# Autodesk Inventor assembly: ASY NDM 11.0 перегородка
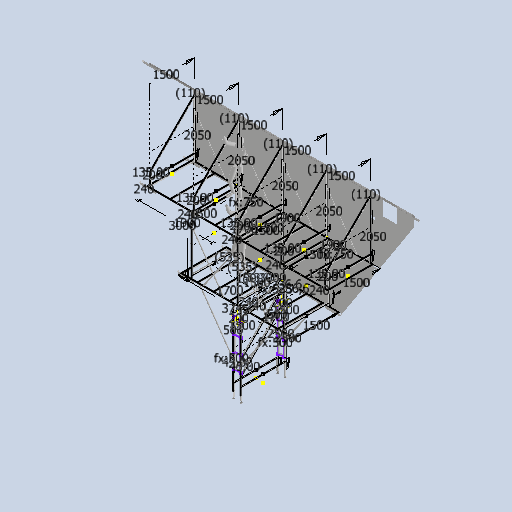
[picture p0: Inventor's stored thumbnail of the model, 512x512]
Saved by Autodesk Inventor 2025 (Build 290162010, 162A)
## iProperties
Created: 2024-05-21
Part Number: ASY NDM 11.0 перегородка
Document SubType Name: Assembly
Designer: admin
Author: admin
## Documents named in this file (18)
- C:\Users\user\YandexDisk\домашниий пк\Inventor\Nadyim\CAD\Перегородка\ASY NDM 11.0 перегородка.iam
- C:\Users\user\YandexDisk\домашниий пк\Inventor\Nadyim\CAD\dummi\human 01\ч ASY human dummy 01.iam
- C:\Users\user\YandexDisk\домашниий пк\Inventor\Nadyim\CAD\Перегородка\NDM 11.012 лист 12.ipt
- C:\Users\user\YandexDisk\домашниий пк\Inventor\Nadyim\CAD\Перегородка\ASY NDM 11.020 перегородка рама 1 горизонт.iam
- C:\Users\user\YandexDisk\домашниий пк\Inventor\Nadyim\CAD\Перегородка\ASY NDM 11.030 перегородка рама 2 горизонт.iam
- C:\Users\user\YandexDisk\домашниий пк\Inventor\Nadyim\CAD\Перегородка\ASY NDM 11.023 перегородка рама 1 вертикал.iam
- C:\Users\user\YandexDisk\домашниий пк\Inventor\Nadyim\CAD\Screwjack pilar\ASY NDM 14.0 Screwjack pillar 1.iam
- C:\Users\user\YandexDisk\домашниий пк\Inventor\Nadyim\CAD\NDM 7.4 bracket bottom mother.ipt
- C:\Users\user\YandexDisk\домашниий пк\Inventor\Nadyim\CAD\Перегородка\ASY NDM 11.040 рама 3 вертикал угол.iam
- C:\Users\user\YandexDisk\домашниий пк\Inventor\Nadyim\CAD\Перегородка\ASY NDM 11.050 перегородка рама 2 вертикал.iam
- C:\Users\user\YandexDisk\домашниий пк\Inventor\Nadyim\CAD\Перегородка\ASY NDM 11.043 верхняя перемычка.ipt
- C:\Users\user\YandexDisk\домашниий пк\Inventor\Nadyim\CAD\Перегородка\ASY NDM 11.025 перегородка рама 1.1  вертикал.iam
- C:\Users\user\YandexDisk\домашниий пк\Inventor\Nadyim\CAD\Перегородка\ASY NDM 11.035 укосина.iam
- C:\Users\user\YandexDisk\домашниий пк\Inventor\Nadyim\CAD\Перегородка\ASY NDM 11.036 укосина.iam
- C:\Users\user\YandexDisk\домашниий пк\Inventor\Nadyim\CAD\Перегородка\ASY NDM 11.037 упор.iam
- C:\Users\user\YandexDisk\домашниий пк\Inventor\Nadyim\CAD\Перегородка\NDM 11.013 лист 131.ipt
- C:\Users\user\YandexDisk\домашниий пк\Inventor\Nadyim\CAD\Перегородка\NDM 11.014 лист 141.ipt
- C:\Users\user\YandexDisk\домашниий пк\Inventor\Nadyim\CAD\Перегородка\NDM 11.015 лист 15.ipt
## Components (62 placed, 17 different names)
1. ч ASY human dummy 01:1 [sub-assembly]
2. ч ASY human dummy 01:2 [sub-assembly]
3. ASY NDM 11.020 перегородка рама 1 горизонт:1 [sub-assembly] — Mate:3, Flush:4, Flush:6, Flush:8, Mate:8, Flush:10, Mate:25, Mate:31, Mate:34, Mate:35, Mate:36, Mate:68, Mate:72, Mate:77, Mate:80, Mate:82, Flush:14, Mate:84, Mate:85, Mate:88, Mate:89, Mate:96, Mate:97
4. ASY NDM 11.030 перегородка рама 2 горизонт:1 [sub-assembly] — Rigid:16, Mate:6, Flush:7, Flush:8, Mate:10, Mate:43, Mate:49, Mate:61, Mate:62, Mate:83, Flush:15, Mate:86, Mate:87, Mate:107, Mate:108
5. ASY NDM 11.030 перегородка рама 2 горизонт:2 [sub-assembly] — Rigid:16, Mate:7, Mate:40, Mate:50, Mate:51, Mate:56, Mate:92, Mate:93, Mate:94, Mate:95, Mate:104, Mate:105, Mate:112, Mate:113
6. ASY NDM 11.023 перегородка рама 1 вертикал:1 [sub-assembly] — Mate:3, Flush:4, Rigid:19, Rigid:20, Mate:5, Flush:5, Rigid:21, Flush:12, Mate:15, Mate:16, Mate:18, Mate:19, Mate:66, Mate:67, Mate:73, Mate:74
7. ASY NDM 14.0 Screwjack pillar 1:1 [sub-assembly] — Rigid:17, Rigid:20, Mate:4
8. NDM 7.4 bracket bottom mother:1 — Rigid:17
9. ASY NDM 14.0 Screwjack pillar 1:2 [sub-assembly] — Rigid:19
10. NDM 7.4 bracket bottom mother:2
11. ASY NDM 11.023 перегородка рама 1 вертикал:2 [sub-assembly] — Rigid:21, Rigid:28, Rigid:29, Mate:17, Mate:75, Mate:76, Mate:78, Mate:79
12. ASY NDM 11.050 перегородка рама 2 вертикал:1 [sub-assembly] — Mate:8, Flush:10, Mate:9, Mate:10, Rigid:22, Rigid:23, Mate:29, Mate:30, Mate:32, Mate:33, Mate:106, Mate:109
13. ASY NDM 11.050 перегородка рама 2 вертикал:2 [sub-assembly] — Rigid:22, Mate:37
14. ASY NDM 11.050 перегородка рама 2 вертикал:3 [sub-assembly] — Rigid:23, Mate:110, Mate:111, Mate:114
15. ASY NDM 11.043 верхняя перемычка:1 — Rigid:31, Mate:90, Mate:91, Mate:101, Mate:102
16. ASY NDM 11.043 верхняя перемычка:2 — Rigid:30, Rigid:31, Rigid:32, Mate:98, Mate:99
17. ASY NDM 14.0 Screwjack pillar 1:3 [sub-assembly] — Rigid:28
18. NDM 7.4 bracket bottom mother:3
19. ASY NDM 14.0 Screwjack pillar 1:4 [sub-assembly] — Rigid:29
20. NDM 7.4 bracket bottom mother:4
21. ASY NDM 11.025 перегородка рама 1.1  вертикал:1 [sub-assembly] — Flush:12, Mate:15, Mate:16
22. ASY NDM 11.025 перегородка рама 1.1  вертикал:2 [sub-assembly] — Mate:17, Mate:18, Mate:19
23. ASY NDM 11.035 укосина:2 [sub-assembly] — Mate:25, Mate:110, Mate:111
24. ASY NDM 11.035 укосина:3 [sub-assembly] — Mate:44, Mate:45, Mate:50
25. ASY NDM 11.035 укосина:4 [sub-assembly] — Mate:41, Mate:42, Mate:43
26. ASY NDM 11.035 укосина:5 [sub-assembly] — Mate:29, Mate:30, Mate:31
27. ASY NDM 11.036 укосина:1 [sub-assembly] — Mate:32, Mate:33, Mate:34
28. ASY NDM 11.036 укосина:2 [sub-assembly] — Mate:35, Mate:36, Mate:37
29. ASY NDM 11.036 укосина:3 [sub-assembly] — Mate:38, Mate:39, Mate:40
30. ASY NDM 11.035 укосина:6 [sub-assembly] — Mate:51, Mate:52, Mate:53
31. ASY NDM 11.035 укосина:7 [sub-assembly] — Mate:46, Mate:47, Mate:48, Mate:49
32. ASY NDM 11.036 укосина:4 [sub-assembly] — Mate:54, Mate:55, Mate:56
33. ASY NDM 11.036 укосина:5 [sub-assembly] — Mate:57, Mate:58, Mate:62
34. ASY NDM 11.036 укосина:6 [sub-assembly] — Mate:59, Mate:60, Mate:61
35. ASY NDM 11.043 верхняя перемычка:3 — Rigid:32
36. ASY NDM 11.035 укосина:8 [sub-assembly] — Mate:66, Mate:67, Mate:68
37. ASY NDM 11.035 укосина:9 [sub-assembly] — Mate:72, Mate:73, Mate:74
38. ASY NDM 11.035 укосина:10 [sub-assembly] — Mate:75, Mate:76, Mate:77
39. ASY NDM 11.035 укосина:11 [sub-assembly] — Mate:78, Mate:79, Mate:80
40. ASY NDM 11.037 упор:1 [sub-assembly]
41. ASY NDM 11.037 упор:2 [sub-assembly] — Mate:83, Flush:15, Flush:16
42. ASY NDM 11.037 упор:3 [sub-assembly] — Mate:82, Flush:14, Flush:17
43. ASY NDM 11.037 упор:4 [sub-assembly] — Mate:84, Mate:85, Flush:17
44. ASY NDM 11.037 упор:5 [sub-assembly] — Mate:86, Mate:87, Flush:16
45. ASY NDM 11.037 упор:6 [sub-assembly] — Mate:92, Mate:94, Flush:19, Flush:21
46. ASY NDM 11.037 упор:7 [sub-assembly] — Mate:93, Mate:95, Flush:19
47. ASY NDM 11.037 упор:8 [sub-assembly] — Mate:89, Mate:96, Flush:18, Flush:20, Flush:21
48. ASY NDM 11.037 упор:9 [sub-assembly] — Mate:88, Mate:97, Flush:18
49. ASY NDM 11.037 упор:10 [sub-assembly] — Mate:90, Mate:91, Flush:20
50. NDM 11.013 лист 131:1 — Mate:101, Mate:102, Mate:103
51. NDM 11.014 лист 141:1 — Mate:104, Mate:105, Mate:106
52. NDM 11.014 лист 141:2 — Mate:107, Mate:108, Mate:109
53. NDM 11.015 лист 15:1 — Mate:112, Mate:113, Mate:114
54. ASY NDM 11.040 рама 3 вертикал угол:1 [sub-assembly] — Mate:6, Flush:7, Flush:9, Mate:38, Mate:39, Mate:41, Mate:42, Rigid:30
55. ASY NDM 11.040 рама 3 вертикал угол:2 [sub-assembly] — Mate:46, Mate:47, Mate:48, Mate:57, Mate:58
56. ASY NDM 11.040 рама 3 вертикал угол:3 [sub-assembly] — Mate:44, Mate:45, Mate:54, Mate:55
57. ASY NDM 11.040 рама 3 вертикал угол:4 [sub-assembly] — Mate:59, Mate:60
58. ASY NDM 11.040 рама 3 вертикал угол:5 [sub-assembly] — Mate:52, Mate:53, Mate:100, Mate:103
59. NDM 11.012 лист 12:5 — Mate:98, Mate:99, Mate:100
60. NDM 11.012 лист 12:6
61. NDM 11.012 лист 12:7
62. NDM 11.012 лист 12:8
## Component patterns: (5 elements, first: ASY NDM 11.040 рама 3 вертикал угол:1), (4 elements, first: NDM 11.012 лист 12:5)
## Relationships (126: Mate 94, Flush 17, WeldJoint 15)
- Rigid:16 [WeldJoint]: ASY NDM 11.030 перегородка рама 2 горизонт:1 ↔ ASY NDM 11.030 перегородка рама 2 горизонт:2
- Mate:3: ASY NDM 11.020 перегородка рама 1 горизонт:1 ↔ ASY NDM 11.023 перегородка рама 1 вертикал:1
- Flush:4: ASY NDM 11.020 перегородка рама 1 горизонт:1 ↔ ASY NDM 11.023 перегородка рама 1 вертикал:1
- Rigid:17 [WeldJoint] (40 mm): ASY NDM 14.0 Screwjack pillar 1:1 ↔ NDM 7.4 bracket bottom mother:1
- [WeldJoint] (40 mm): ASY NDM 14.0 Screwjack pillar 1:2 ↔ NDM 7.4 bracket bottom mother:2
- Rigid:19 [WeldJoint]: ASY NDM 11.023 перегородка рама 1 вертикал:1 ↔ ASY NDM 14.0 Screwjack pillar 1:2
- Rigid:20 [WeldJoint]: ASY NDM 11.023 перегородка рама 1 вертикал:1 ↔ ASY NDM 14.0 Screwjack pillar 1:1
- Mate:4: ASY NDM 14.0 Screwjack pillar 1:1
- Mate:5 (100 mm): ASY NDM 11.023 перегородка рама 1 вертикал:1
- Flush:5: ASY NDM 11.023 перегородка рама 1 вертикал:1
- Flush:6: ASY NDM 11.020 перегородка рама 1 горизонт:1
- Mate:6: ASY NDM 11.030 перегородка рама 2 горизонт:1 ↔ ASY NDM 11.040 рама 3 вертикал угол:1
- Flush:7: ASY NDM 11.030 перегородка рама 2 горизонт:1 ↔ ASY NDM 11.040 рама 3 вертикал угол:1
- Rigid:21 [WeldJoint] (204 mm): ASY NDM 11.023 перегородка рама 1 вертикал:1 ↔ ASY NDM 11.023 перегородка рама 1 вертикал:2
- Flush:8: ASY NDM 11.020 перегородка рама 1 горизонт:1 ↔ ASY NDM 11.030 перегородка рама 2 горизонт:1
- Flush:9: ASY NDM 11.040 рама 3 вертикал угол:1
- Mate:7: ASY NDM 11.030 перегородка рама 2 горизонт:2
- Mate:8 (2 mm): ASY NDM 11.020 перегородка рама 1 горизонт:1 ↔ ASY NDM 11.050 перегородка рама 2 вертикал:1
- Flush:10: ASY NDM 11.020 перегородка рама 1 горизонт:1 ↔ ASY NDM 11.050 перегородка рама 2 вертикал:1
- Mate:9: ASY NDM 11.050 перегородка рама 2 вертикал:1
- Mate:10 (2 mm): ASY NDM 11.030 перегородка рама 2 горизонт:1 ↔ ASY NDM 11.050 перегородка рама 2 вертикал:1
- Rigid:22 [WeldJoint] (1490 mm): ASY NDM 11.050 перегородка рама 2 вертикал:1 ↔ ASY NDM 11.050 перегородка рама 2 вертикал:2
- Rigid:23 [WeldJoint] (1530 mm): ASY NDM 11.050 перегородка рама 2 вертикал:1 ↔ ASY NDM 11.050 перегородка рама 2 вертикал:3
- [WeldJoint] (40 mm): ASY NDM 14.0 Screwjack pillar 1:3 ↔ NDM 7.4 bracket bottom mother:3
- [WeldJoint] (40 mm): ASY NDM 14.0 Screwjack pillar 1:4 ↔ NDM 7.4 bracket bottom mother:4
- Rigid:28 [WeldJoint]: ASY NDM 11.023 перегородка рама 1 вертикал:2 ↔ ASY NDM 14.0 Screwjack pillar 1:3
- Rigid:29 [WeldJoint]: ASY NDM 11.023 перегородка рама 1 вертикал:2 ↔ ASY NDM 14.0 Screwjack pillar 1:4
- Flush:12: ASY NDM 11.023 перегородка рама 1 вертикал:1 ↔ ASY NDM 11.025 перегородка рама 1.1  вертикал:1
- Mate:15: ASY NDM 11.023 перегородка рама 1 вертикал:1 ↔ ASY NDM 11.025 перегородка рама 1.1  вертикал:1
- Mate:16 (100 mm): ASY NDM 11.023 перегородка рама 1 вертикал:1 ↔ ASY NDM 11.025 перегородка рама 1.1  вертикал:1
- Mate:17: ASY NDM 11.023 перегородка рама 1 вертикал:2 ↔ ASY NDM 11.025 перегородка рама 1.1  вертикал:2
- Mate:18 (100 mm): ASY NDM 11.023 перегородка рама 1 вертикал:1 ↔ ASY NDM 11.025 перегородка рама 1.1  вертикал:2
- Mate:19: ASY NDM 11.023 перегородка рама 1 вертикал:1 ↔ ASY NDM 11.025 перегородка рама 1.1  вертикал:2
- Mate:25: ASY NDM 11.020 перегородка рама 1 горизонт:1 ↔ ASY NDM 11.035 укосина:2
- Mate:29: ASY NDM 11.050 перегородка рама 2 вертикал:1 ↔ ASY NDM 11.035 укосина:5
- Mate:30: ASY NDM 11.050 перегородка рама 2 вертикал:1 ↔ ASY NDM 11.035 укосина:5
- Mate:31: ASY NDM 11.020 перегородка рама 1 горизонт:1 ↔ ASY NDM 11.035 укосина:5
- Mate:32: ASY NDM 11.050 перегородка рама 2 вертикал:1 ↔ ASY NDM 11.036 укосина:1
- Mate:33: ASY NDM 11.050 перегородка рама 2 вертикал:1 ↔ ASY NDM 11.036 укосина:1
- Mate:34: ASY NDM 11.020 перегородка рама 1 горизонт:1 ↔ ASY NDM 11.036 укосина:1
- Mate:35: ASY NDM 11.020 перегородка рама 1 горизонт:1 ↔ ASY NDM 11.036 укосина:2
- Mate:36: ASY NDM 11.020 перегородка рама 1 горизонт:1 ↔ ASY NDM 11.036 укосина:2
- Mate:37: ASY NDM 11.050 перегородка рама 2 вертикал:2 ↔ ASY NDM 11.036 укосина:2
- Mate:38: ASY NDM 11.036 укосина:3 ↔ ASY NDM 11.040 рама 3 вертикал угол:1
- Mate:39: ASY NDM 11.036 укосина:3 ↔ ASY NDM 11.040 рама 3 вертикал угол:1
- Mate:40: ASY NDM 11.030 перегородка рама 2 горизонт:2 ↔ ASY NDM 11.036 укосина:3
- Mate:41: ASY NDM 11.035 укосина:4 ↔ ASY NDM 11.040 рама 3 вертикал угол:1
- Mate:42: ASY NDM 11.035 укосина:4 ↔ ASY NDM 11.040 рама 3 вертикал угол:1
- Mate:43: ASY NDM 11.030 перегородка рама 2 горизонт:1 ↔ ASY NDM 11.035 укосина:4
- Mate:44: ASY NDM 11.035 укосина:3 ↔ ASY NDM 11.040 рама 3 вертикал угол:3
- Mate:45: ASY NDM 11.035 укосина:3 ↔ ASY NDM 11.040 рама 3 вертикал угол:3
- Mate:46: ASY NDM 11.035 укосина:7 ↔ ASY NDM 11.040 рама 3 вертикал угол:2
- Mate:47: ASY NDM 11.035 укосина:7 ↔ ASY NDM 11.040 рама 3 вертикал угол:2
- Mate:48: ASY NDM 11.035 укосина:7 ↔ ASY NDM 11.040 рама 3 вертикал угол:2
- Mate:49: ASY NDM 11.030 перегородка рама 2 горизонт:1 ↔ ASY NDM 11.035 укосина:7
- Mate:50: ASY NDM 11.030 перегородка рама 2 горизонт:2 ↔ ASY NDM 11.035 укосина:3
- Mate:51: ASY NDM 11.030 перегородка рама 2 горизонт:2 ↔ ASY NDM 11.035 укосина:6
- Mate:52: ASY NDM 11.035 укосина:6 ↔ ASY NDM 11.040 рама 3 вертикал угол:5
- Mate:53: ASY NDM 11.035 укосина:6 ↔ ASY NDM 11.040 рама 3 вертикал угол:5
- Rigid:30 [WeldJoint]: ASY NDM 11.043 верхняя перемычка:2 ↔ ASY NDM 11.040 рама 3 вертикал угол:1
- Mate:54: ASY NDM 11.036 укосина:4 ↔ ASY NDM 11.040 рама 3 вертикал угол:3
- Mate:55: ASY NDM 11.036 укосина:4 ↔ ASY NDM 11.040 рама 3 вертикал угол:3
- Mate:56: ASY NDM 11.030 перегородка рама 2 горизонт:2 ↔ ASY NDM 11.036 укосина:4
- Mate:57: ASY NDM 11.036 укосина:5 ↔ ASY NDM 11.040 рама 3 вертикал угол:2
- Mate:58: ASY NDM 11.036 укосина:5 ↔ ASY NDM 11.040 рама 3 вертикал угол:2
- Mate:59: ASY NDM 11.036 укосина:6 ↔ ASY NDM 11.040 рама 3 вертикал угол:4
- Mate:60: ASY NDM 11.036 укосина:6 ↔ ASY NDM 11.040 рама 3 вертикал угол:4
- Mate:61: ASY NDM 11.030 перегородка рама 2 горизонт:1 ↔ ASY NDM 11.036 укосина:6
- Mate:62: ASY NDM 11.030 перегородка рама 2 горизонт:1 ↔ ASY NDM 11.036 укосина:5
- Rigid:31 [WeldJoint]: ASY NDM 11.043 верхняя перемычка:1 ↔ ASY NDM 11.043 верхняя перемычка:2
- Rigid:32 [WeldJoint]: ASY NDM 11.043 верхняя перемычка:2 ↔ ASY NDM 11.043 верхняя перемычка:3
- Mate:66: ASY NDM 11.023 перегородка рама 1 вертикал:1 ↔ ASY NDM 11.035 укосина:8
- Mate:67: ASY NDM 11.023 перегородка рама 1 вертикал:1 ↔ ASY NDM 11.035 укосина:8
- Mate:68: ASY NDM 11.020 перегородка рама 1 горизонт:1 ↔ ASY NDM 11.035 укосина:8
- Mate:72: ASY NDM 11.020 перегородка рама 1 горизонт:1 ↔ ASY NDM 11.035 укосина:9
- Mate:73: ASY NDM 11.023 перегородка рама 1 вертикал:1 ↔ ASY NDM 11.035 укосина:9
- Mate:74: ASY NDM 11.023 перегородка рама 1 вертикал:1 ↔ ASY NDM 11.035 укосина:9
- Mate:75: ASY NDM 11.023 перегородка рама 1 вертикал:2 ↔ ASY NDM 11.035 укосина:10
- Mate:76: ASY NDM 11.023 перегородка рама 1 вертикал:2 ↔ ASY NDM 11.035 укосина:10
- Mate:77: ASY NDM 11.020 перегородка рама 1 горизонт:1 ↔ ASY NDM 11.035 укосина:10
- Mate:78: ASY NDM 11.023 перегородка рама 1 вертикал:2 ↔ ASY NDM 11.035 укосина:11
- Mate:79: ASY NDM 11.023 перегородка рама 1 вертикал:2 ↔ ASY NDM 11.035 укосина:11
- Mate:80: ASY NDM 11.020 перегородка рама 1 горизонт:1 ↔ ASY NDM 11.035 укосина:11
- [Mate]: ASY NDM 11.043 верхняя перемычка:3 ↔ ASY NDM 11.037 упор:1
- [Flush]: ASY NDM 11.043 верхняя перемычка:3 ↔ ASY NDM 11.037 упор:1
- Mate:82: ASY NDM 11.020 перегородка рама 1 горизонт:1 ↔ ASY NDM 11.037 упор:3
- Flush:14: ASY NDM 11.020 перегородка рама 1 горизонт:1 ↔ ASY NDM 11.037 упор:3
- Mate:83: ASY NDM 11.030 перегородка рама 2 горизонт:1 ↔ ASY NDM 11.037 упор:2
- Flush:15: ASY NDM 11.030 перегородка рама 2 горизонт:1 ↔ ASY NDM 11.037 упор:2
- Mate:84: ASY NDM 11.020 перегородка рама 1 горизонт:1 ↔ ASY NDM 11.037 упор:4
- Mate:85: ASY NDM 11.020 перегородка рама 1 горизонт:1 ↔ ASY NDM 11.037 упор:4
- Mate:86: ASY NDM 11.030 перегородка рама 2 горизонт:1 ↔ ASY NDM 11.037 упор:5
- Mate:87: ASY NDM 11.030 перегородка рама 2 горизонт:1 ↔ ASY NDM 11.037 упор:5
- Flush:16: ASY NDM 11.037 упор:2 ↔ ASY NDM 11.037 упор:5
- Flush:17: ASY NDM 11.037 упор:3 ↔ ASY NDM 11.037 упор:4
- Mate:88: ASY NDM 11.020 перегородка рама 1 горизонт:1 ↔ ASY NDM 11.037 упор:9
- Mate:89: ASY NDM 11.020 перегородка рама 1 горизонт:1 ↔ ASY NDM 11.037 упор:8
- Mate:90: ASY NDM 11.043 верхняя перемычка:1 ↔ ASY NDM 11.037 упор:10
- Mate:91: ASY NDM 11.043 верхняя перемычка:1 ↔ ASY NDM 11.037 упор:10
- Mate:92: ASY NDM 11.030 перегородка рама 2 горизонт:2 ↔ ASY NDM 11.037 упор:6
- Mate:93: ASY NDM 11.030 перегородка рама 2 горизонт:2 ↔ ASY NDM 11.037 упор:7
- Mate:94: ASY NDM 11.030 перегородка рама 2 горизонт:2 ↔ ASY NDM 11.037 упор:6
- Mate:95: ASY NDM 11.030 перегородка рама 2 горизонт:2 ↔ ASY NDM 11.037 упор:7
- Mate:96: ASY NDM 11.020 перегородка рама 1 горизонт:1 ↔ ASY NDM 11.037 упор:8
- Mate:97: ASY NDM 11.020 перегородка рама 1 горизонт:1 ↔ ASY NDM 11.037 упор:9
- Flush:18: ASY NDM 11.037 упор:8 ↔ ASY NDM 11.037 упор:9
- Flush:19: ASY NDM 11.037 упор:6 ↔ ASY NDM 11.037 упор:7
- Mate:98: ASY NDM 11.043 верхняя перемычка:2 ↔ NDM 11.012 лист 12:5
- Mate:99: ASY NDM 11.043 верхняя перемычка:2 ↔ NDM 11.012 лист 12:5
- Mate:100: ASY NDM 11.040 рама 3 вертикал угол:5 ↔ NDM 11.012 лист 12:5
- Mate:101: ASY NDM 11.043 верхняя перемычка:1 ↔ NDM 11.013 лист 131:1
- Mate:102: ASY NDM 11.043 верхняя перемычка:1 ↔ NDM 11.013 лист 131:1
- Mate:103: NDM 11.013 лист 131:1 ↔ ASY NDM 11.040 рама 3 вертикал угол:5
- Flush:20: ASY NDM 11.037 упор:8 ↔ ASY NDM 11.037 упор:10
- Flush:21: ASY NDM 11.037 упор:6 ↔ ASY NDM 11.037 упор:8
- Mate:104: ASY NDM 11.030 перегородка рама 2 горизонт:2 ↔ NDM 11.014 лист 141:1
- Mate:105: ASY NDM 11.030 перегородка рама 2 горизонт:2 ↔ NDM 11.014 лист 141:1
- Mate:106: ASY NDM 11.050 перегородка рама 2 вертикал:1 ↔ NDM 11.014 лист 141:1
- Mate:107: ASY NDM 11.030 перегородка рама 2 горизонт:1 ↔ NDM 11.014 лист 141:2
- Mate:108: ASY NDM 11.030 перегородка рама 2 горизонт:1 ↔ NDM 11.014 лист 141:2
- Mate:109: ASY NDM 11.050 перегородка рама 2 вертикал:1 ↔ NDM 11.014 лист 141:2
- Mate:110: ASY NDM 11.050 перегородка рама 2 вертикал:3 ↔ ASY NDM 11.035 укосина:2
- Mate:111: ASY NDM 11.050 перегородка рама 2 вертикал:3 ↔ ASY NDM 11.035 укосина:2
- Mate:112: ASY NDM 11.030 перегородка рама 2 горизонт:2 ↔ NDM 11.015 лист 15:1
- Mate:113: ASY NDM 11.030 перегородка рама 2 горизонт:2 ↔ NDM 11.015 лист 15:1
- Mate:114: ASY NDM 11.050 перегородка рама 2 вертикал:3 ↔ NDM 11.015 лист 15:1
## Named parameters: МежлистовоеX = 22 mm, МежлистовоеY = 22 mm, d37_d36 = 40 mm, d74_d36 = 40 mm, d75_d36 = 40 mm
